# Autodesk Inventor assembly: ASM_Micron_Rev2_ASAP
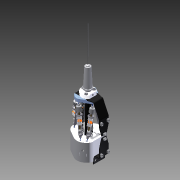
[picture p0: Inventor's stored thumbnail of the model, 180x180]
Saved by Autodesk Inventor 2011 SP2 (Build 150309200, 309)
## iProperties
Created: 2012-01-18
Part Number: ASM_Micron_Rev2_ASAP
Document SubType Name: Assembly
Designer: sungwook
Author: sungwook
## Documents named in this file (11)
- C:\Users\sungwook\Documents\Inventor\Micron20\Assembly\ASM_Micron_Rev2_ASAP-2.iam
- C:\Users\sungwook\Documents\Inventor\Micron20\Parts\Main\Platfrom_Base_20mm_Rev_2.ipt
- C:\Users\sungwook\Documents\Inventor\Micron20\Parts\Main\Platfrom_Top_14mm_Rev_2.ipt
- C:\Users\sungwook\Documents\Inventor\Micron20\Parts\Tool\ASM_Tool_Tip_Rev.iam
- C:\Users\sungwook\Documents\Inventor\Micron20\Assembly\ASM_Motor_Unit_Rev.iam
- C:\Users\sungwook\Documents\Inventor\Micron20\Parts\Main\Eye_Pin_26Ga.ipt
- C:\Users\sungwook\Documents\Inventor\Content Center Files\R2011\en-US\ANSI B18.6.3(12)\ANSI B18.6.3 - 0-80 UNF - 0.1875(15_).ipt
- C:\Users\sungwook\Documents\Inventor\Micron20\Parts\Main\Spring.ipt
- C:\Users\sungwook\Documents\Inventor\Micron20\Parts\ASAP\Handle_ASAP.iam
- C:\Users\sungwook\Documents\Inventor\Micron20\Parts\ASAP\Platform_ASAP.iam
- C:\Users\sungwook\Documents\Inventor\Micron20\Parts\Main\Guide Tube.ipt
## Components (24 placed, 10 different names)
1. Platfrom_Base_20mm_Rev_2:1 — Mate:4, Mate:6, Mate:8, Angle:1, Mate:13, Mate:14, Mate:15, Mate:19, Mate:20
2. Platfrom_Top_14mm_Rev_2:1 — Mate:1, Mate:2, Mate:3, Mate:4, Mate:5, Mate:7, Angle:1, Mate:9, Mate:10, Mate:18
3. ASM_Tool_Tip_Rev:1 [sub-assembly] — Mate:1, Mate:2, Mate:3, Mate:11, Mate:21
4. Handle_ASAP:1 [sub-assembly] — Mate:19, Flush:1
5. Platform_ASAP:1 [sub-assembly] — Mate:16, Mate:17, Mate:18, Mate:22
6. Guide Tube:1 — Mate:21, Mate:22
7. ASM_Motor_Unit_Rev:1 [sub-assembly] — Mate:5, Mate:6
8. ASM_Motor_Unit_Rev:2 [sub-assembly] — Mate:7, Mate:8
9. ASM_Motor_Unit_Rev:3 [sub-assembly]
10. ASM_Motor_Unit_Rev:4 [sub-assembly]
11. ASM_Motor_Unit_Rev:5 [sub-assembly]
12. ASM_Motor_Unit_Rev:6 [sub-assembly]
13. Eye_Pin_26Ga:1 — Mate:9, Mate:10, Mate:12, Angle:2
14. Eye_Pin_26Ga:2
15. Eye_Pin_26Ga:3
16. Cross Recessed Flat Countersunk Head Machine Screw - Type I - Inch 0-80 x 3/16:1 — Mate:11, Mate:16
17. Cross Recessed Flat Countersunk Head Machine Screw - Type I - Inch 0-80 x 3/16:2
18. Cross Recessed Flat Countersunk Head Machine Screw - Type I - Inch 0-80 x 3/16:3 — Mate:17
19. Spring:1 — Mate:12, Mate:13, Mate:20
20. Spring:2
21. Spring:3
22. Eye_Pin_26Ga:4 — Mate:14, Mate:15
23. Eye_Pin_26Ga:5
24. Eye_Pin_26Ga:6
## Component patterns: (3 elements, first: ASM_Motor_Unit_Rev:1 + ASM_Motor_Unit_Rev:2), Eye Pin Top (3 elements), Tool Mount Bolts (3 elements), Springs (3 elements), Eye Pin Bottom (3 elements)
## Relationships (25: Mate 22, Angle 2, Flush 1)
- Mate:1: Platfrom_Top_14mm_Rev_2:1 ↔ ASM_Tool_Tip_Rev:1
- Mate:2: Platfrom_Top_14mm_Rev_2:1 ↔ ASM_Tool_Tip_Rev:1
- Mate:3: Platfrom_Top_14mm_Rev_2:1 ↔ ASM_Tool_Tip_Rev:1
- Mate:4: Platfrom_Base_20mm_Rev_2:1 ↔ Platfrom_Top_14mm_Rev_2:1
- Mate:5: Platfrom_Top_14mm_Rev_2:1 ↔ ASM_Motor_Unit_Rev:1
- Mate:6: Platfrom_Base_20mm_Rev_2:1 ↔ ASM_Motor_Unit_Rev:1
- Mate:7: Platfrom_Top_14mm_Rev_2:1 ↔ ASM_Motor_Unit_Rev:2
- Mate:8: Platfrom_Base_20mm_Rev_2:1 ↔ ASM_Motor_Unit_Rev:2
- Angle:1 (180 deg): Platfrom_Base_20mm_Rev_2:1 ↔ Platfrom_Top_14mm_Rev_2:1
- Mate:9: Platfrom_Top_14mm_Rev_2:1 ↔ Eye_Pin_26Ga:1
- Mate:10: Platfrom_Top_14mm_Rev_2:1 ↔ Eye_Pin_26Ga:1
- Mate:12: Eye_Pin_26Ga:1 ↔ Spring:1
- Mate:13: Platfrom_Base_20mm_Rev_2:1 ↔ Spring:1
- Mate:14: Platfrom_Base_20mm_Rev_2:1 ↔ Eye_Pin_26Ga:4
- Mate:15: Platfrom_Base_20mm_Rev_2:1 ↔ Eye_Pin_26Ga:4
- Mate:16: Platform_ASAP:1 ↔ Cross Recessed Flat Countersunk Head Machine Screw - Type I - Inch 0-80 x 3/16:1
- Mate:17: Platform_ASAP:1 ↔ Cross Recessed Flat Countersunk Head Machine Screw - Type I - Inch 0-80 x 3/16:3
- Mate:18: Platfrom_Top_14mm_Rev_2:1 ↔ Platform_ASAP:1
- Mate:19: Platfrom_Base_20mm_Rev_2:1 ↔ Handle_ASAP:1
- Flush:1: Handle_ASAP:1
- Angle:2 (0 deg): Eye_Pin_26Ga:1
- Mate:20: Platfrom_Base_20mm_Rev_2:1 ↔ Spring:1
- Mate:21: ASM_Tool_Tip_Rev:1 ↔ Guide Tube:1
- Mate:22: Platform_ASAP:1 ↔ Guide Tube:1
- Mate:11: ASM_Tool_Tip_Rev:1 ↔ Cross Recessed Flat Countersunk Head Machine Screw - Type I - Inch 0-80 x 3/16:1
